# Autodesk Inventor assembly: ArmAssembly
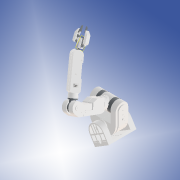
[picture p0: Inventor's stored thumbnail of the model, 180x180]
Saved by Autodesk Inventor 2017 (Build 210142000, 142)
## iProperties
Created: 2017-05-10
Part Number: ArmAssembly
Document SubType Name: Assembly
Designer: zallen
Author: zallen
## Documents named in this file (6)
- C:\Users\zallen\Documents\GitHub\cr-laundry-robot\src\Body\Arm Assembly\ArmAssembly.iam
- C:\Users\zallen\Documents\GitHub\cr-laundry-robot\src\Body\Arm Assembly\Shoulder Joint Assembly\Shoulder Joint Assembly.iam
- C:\Users\zallen\Documents\GitHub\cr-laundry-robot\src\Body\Arm Assembly\Bicep Assembly\BicepAssembly.iam
- C:\Users\zallen\Documents\GitHub\cr-laundry-robot\src\Body\Arm Assembly\Fore Arm Assembly\ForeArmAssembly.iam
- C:\Users\zallen\Documents\GitHub\cr-laundry-robot\src\Body\Arm Assembly\Gripper Assembly\Gripper Assembly.iam
- C:\Users\zallen\Documents\GitHub\cr-laundry-robot\lib\Strain Wave Gearbox 12_1\StrainWaveGearbox_12_1.iam
## Components (5 placed, 5 different names)
1. Shoulder Joint Assembly:1 [sub-assembly] — Mate:67, Mate:68, Mate:69, Mate:77, Mate:79
2. BicepAssembly:1 [sub-assembly] — Mate:77, Mate:79, Mate:80, Mate:81, Mate:82
3. ForeArmAssembly:1 [sub-assembly] — Mate:75, Mate:76, Mate:83, Mate:84
4. Gripper Assembly:1 [sub-assembly] — Mate:75, Mate:76
5. StrainWaveGearbox_12_1:1 [sub-assembly] — Mate:80, Mate:81, Mate:82, Mate:83, Mate:84
## Relationships (12: Mate 12)
- Mate:67: Shoulder Joint Assembly:1
- Mate:68: Shoulder Joint Assembly:1
- Mate:69: Shoulder Joint Assembly:1
- Mate:75: ForeArmAssembly:1 ↔ Gripper Assembly:1
- Mate:76: ForeArmAssembly:1 ↔ Gripper Assembly:1
- Mate:77: Shoulder Joint Assembly:1 ↔ BicepAssembly:1
- Mate:79: Shoulder Joint Assembly:1 ↔ BicepAssembly:1
- Mate:80: BicepAssembly:1 ↔ StrainWaveGearbox_12_1:1
- Mate:81: BicepAssembly:1 ↔ StrainWaveGearbox_12_1:1
- Mate:82: BicepAssembly:1 ↔ StrainWaveGearbox_12_1:1
- Mate:83: ForeArmAssembly:1 ↔ StrainWaveGearbox_12_1:1
- Mate:84: ForeArmAssembly:1 ↔ StrainWaveGearbox_12_1:1
